# Autodesk Inventor assembly: SideWheel
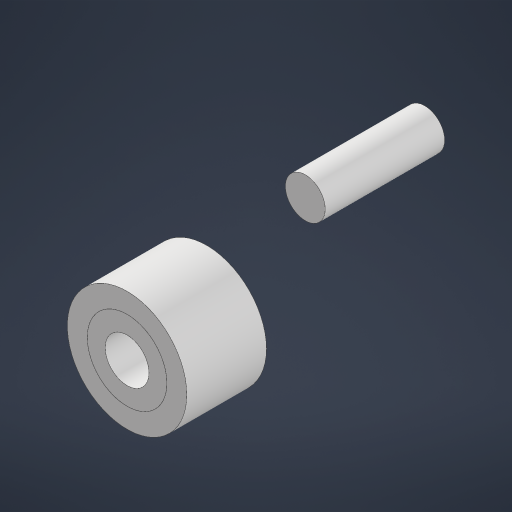
[picture p0: Inventor's stored thumbnail of the model, 512x512]
Saved by Autodesk Inventor 2024.2 (Build 282272000, 272)
## iProperties
Created: 2023-12-20
Part Number: SideWheel
Document SubType Name: Assembly
Designer: Hanaoka
Author: Hanaoka
## Documents named in this file (4)
- G:\共有ドライブ\reRo\05_個人\hanaoka\inventor\SideWheel.iam
- G:\共有ドライブ\reRo\05_個人\hanaoka\inventor\SiliconeTube_6x4x4.ipt
- G:\共有ドライブ\reRo\05_個人\hanaoka\inventor\Spacer_4x2x4.ipt
- G:\共有ドライブ\reRo\05_個人\hanaoka\inventor\NockPin_2x6.ipt
## Components (3 placed, 3 different names)
1. SiliconeTube_6x4x4:1 — 挿入:1
2. Spacer_4x2x4:1 — 挿入:1
3. NockPin_2x6:1
## Relationships (1: Insert 1)
- 挿入:1 [Insert]: SiliconeTube_6x4x4:1 ↔ Spacer_4x2x4:1
